# Autodesk Inventor assembly: manipulator_asembly
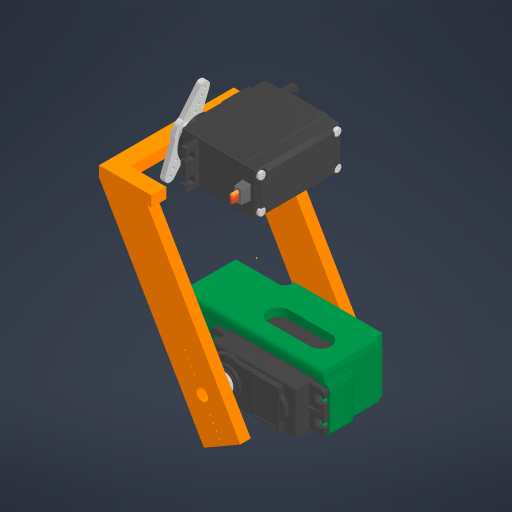
[picture p0: Inventor's stored thumbnail of the model, 512x512]
Saved by Autodesk Inventor 2024 (Build 280153000, 153)
## iProperties
Created: 2023-05-17
Part Number: manipulator_asembly
Document SubType Name: Assembly
Designer: user
Author: user
## Documents named in this file (4)
- D:\Docs\Robot\3d\manipulator\manipulator_asembly.iam
- D:\Docs\Robot\3d\manipulator\manipulator_asembly\manipulator_holder.ipt
- D:\Docs\Robot\3d\electronics\servo\MG996R SBORKA.iam
- D:\Docs\Robot\3d\manipulator\manipulator_asembly\manipulator_arm.ipt
## Components (4 placed, 3 different names)
1. manipulator_holder:1 — Заподлицо:1, Заподлицо:2, Совмещение:1, Совмещение:3, Совмещение:4, Совмещение:5, Заподлицо:4, Заподлицо:5
2. MG996R SBORKA:1 [sub-assembly] — Совмещение:3, Совмещение:4, Совмещение:5, Заподлицо:3
3. manipulator_arm:1 — Заподлицо:3, Заподлицо:4, Заподлицо:5, Совмещение:7
4. MG996R SBORKA:2 [sub-assembly] — Совмещение:7
## Relationships (10: Flush 5, Mate 5)
- Заподлицо:1 [Flush]: manipulator_holder:1
- Заподлицо:2 [Flush]: manipulator_holder:1
- Совмещение:1 [Mate]: manipulator_holder:1
- Совмещение:3 [Mate]: manipulator_holder:1 ↔ MG996R SBORKA:1
- Совмещение:4 [Mate]: manipulator_holder:1 ↔ MG996R SBORKA:1
- Совмещение:5 [Mate]: manipulator_holder:1 ↔ MG996R SBORKA:1
- Заподлицо:3 [Flush]: MG996R SBORKA:1 ↔ manipulator_arm:1
- Заподлицо:4 [Flush]: manipulator_holder:1 ↔ manipulator_arm:1
- Заподлицо:5 [Flush]: manipulator_holder:1 ↔ manipulator_arm:1
- Совмещение:7 [Mate] (3 mm): manipulator_arm:1 ↔ MG996R SBORKA:2
